# Autodesk Inventor assembly: Эксперемент листы бака Глеб
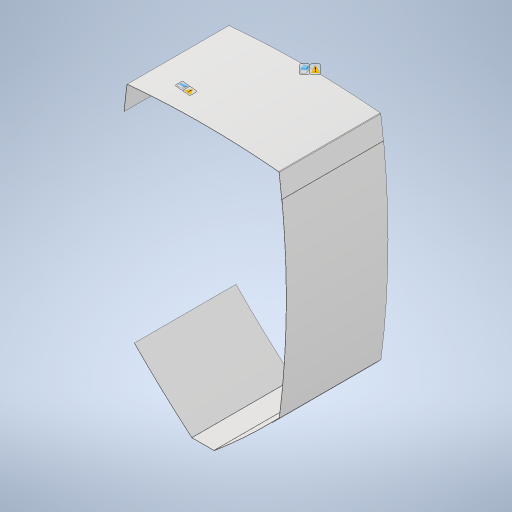
[picture p0: Inventor's stored thumbnail of the model, 512x512]
Saved by Autodesk Inventor 2024.2 (Build 282272000, 272)
## iProperties
Created: 2024-06-02
Part Number: Эксперемент листы бака Глеб
Document SubType Name: Assembly
Designer: pokla
Author: pokla
## Documents named in this file (5)
- C:\Users\pokla\Documents\Inventor\Отстойник осветлитель\Manturovo_Se-clar-Gleb\Листы бака Глеб\Эксперемент листы бака Глеб.iam
- C:\Users\pokla\Documents\Inventor\Отстойник осветлитель\Manturovo_Se-clar-Gleb\Листы бака Глеб\МОО 010 лист спина 1 Глеб.ipt
- C:\Users\pokla\Documents\Inventor\Отстойник осветлитель\Manturovo_Se-clar-Gleb\Листы бака Глеб\МОО 020 лист борт 1  Глеб.ipt
- C:\Users\pokla\Documents\Inventor\Отстойник осветлитель\Manturovo_Se-clar-Gleb\Листы бака Глеб\МОО 030 лист брюхо 1  Глеб.ipt
- C:\Users\pokla\Documents\Inventor\Отстойник осветлитель\Manturovo_Se-clar-Gleb\Листы бака Глеб\МОО 020 лист борт 1  Глеб_CPY.ipt
## Components (4 placed, 4 different names)
1. МОО 010 лист спина 1 Глеб:1 — Mate:1, Flush:1, Mate:2, Rigid:1, Rigid:2
2. МОО 020 лист борт 1  Глеб:1 — Rigid:1
3. МОО 030 лист брюхо 1  Глеб:1 — Rigid:3
4. МОО 020 лист борт 1  Глеб_CPY:1 — Rigid:2, Rigid:3
## Relationships (6: WeldJoint 3, Mate 2, Flush 1)
- Mate:1: МОО 010 лист спина 1 Глеб:1
- Flush:1: МОО 010 лист спина 1 Глеб:1
- Mate:2: МОО 010 лист спина 1 Глеб:1
- Rigid:1 [WeldJoint]: МОО 010 лист спина 1 Глеб:1 ↔ МОО 020 лист борт 1  Глеб:1
- Rigid:2 [WeldJoint]: МОО 010 лист спина 1 Глеб:1 ↔ МОО 020 лист борт 1  Глеб_CPY:1
- Rigid:3 [WeldJoint]: МОО 030 лист брюхо 1  Глеб:1 ↔ МОО 020 лист борт 1  Глеб_CPY:1
